# Autodesk Inventor assembly: Joining Plate T-Type for 4040 A
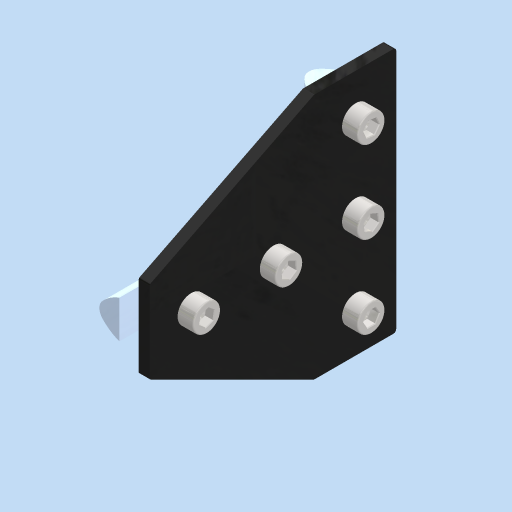
[picture p0: Inventor's stored thumbnail of the model, 512x512]
Saved by Autodesk Inventor 2023.2 (Build 272271000, 271)
## iProperties
Created: 2023-11-29
Part Number: Joining Plate T-Type for 4040 A
Document SubType Name: Assembly
Designer: Nils Bade
Author: Nils Bade
## Documents named in this file (5)
- C:\Users\nilsb\Documents\Inventor\Projektarbeit-Bade\RatRig_modified\Joining Plate T-Type for 4040 A - ItemNuts.iam
- C:\Users\nilsb\Documents\Inventor\Projektarbeit-Bade\RatRig_Standards\Joining Plate for 3030 - T - Black Anodized v2.ipt
- C:\Users\nilsb\Documents\Inventor\Projektarbeit-Bade\Schrauben\Cap Head Screw M6x12 v2.ipt
- C:\Users\nilsb\Documents\Inventor\Projektarbeit-Bade\ITEM\item_Nutenstein 8 - M6_0002623.ipt
- item_Nutenstein 8 - M6_0002623.ipt
## Components (11 placed, 3 different names)
1. Joining Plate for 3030 - T - Black Anodized v2:1 — Passend:1, Passend:2, Passend:3, Passend:4, Passend:5, Passend:6, Passend:7, Passend:8, Passend:9, Passend:10, Winkel:1, Winkel:2, Winkel:3, Winkel:4, Winkel:5, Passend:30, Passend:31, Passend:32, Passend:33, Passend:34
2. Cap Head Screw M6x12 v2:1 — Passend:1, Passend:7, Passend:26
3. Cap Head Screw M6x12 v2:2 — Passend:2, Passend:8, Passend:25
4. Cap Head Screw M6x12 v2:3 — Passend:3, Passend:6, Passend:29
5. Cap Head Screw M6x12 v2:4 — Passend:4, Passend:9, Passend:22, Passend:27
6. Cap Head Screw M6x12 v2:5 — Passend:5, Passend:10, Passend:21, Passend:28
7. item_Nutenstein 8 - M6_0002623:1 — Passend:28, Winkel:3, Passend:34
8. item_Nutenstein 8 - M6_0002623:2 — Passend:27, Winkel:2, Passend:31
9. item_Nutenstein 8 - M6_0002623:3 — Passend:29, Winkel:1, Passend:30
10. item_Nutenstein 8 - M6_0002623:4 — Passend:25, Winkel:4, Passend:32
11. item_Nutenstein 8 - M6_0002623:5 — Passend:26, Winkel:5, Passend:33
## Relationships (30: Mate 24, Angle 5, Flush 1)
- Passend:1 [Mate]: Joining Plate for 3030 - T - Black Anodized v2:1 ↔ Cap Head Screw M6x12 v2:1
- Passend:2 [Mate]: Joining Plate for 3030 - T - Black Anodized v2:1 ↔ Cap Head Screw M6x12 v2:2
- Passend:3 [Mate]: Joining Plate for 3030 - T - Black Anodized v2:1 ↔ Cap Head Screw M6x12 v2:3
- Passend:4 [Mate]: Joining Plate for 3030 - T - Black Anodized v2:1 ↔ Cap Head Screw M6x12 v2:4
- Passend:5 [Mate]: Joining Plate for 3030 - T - Black Anodized v2:1 ↔ Cap Head Screw M6x12 v2:5
- Passend:6 [Mate]: Joining Plate for 3030 - T - Black Anodized v2:1 ↔ Cap Head Screw M6x12 v2:3
- Passend:7 [Mate]: Joining Plate for 3030 - T - Black Anodized v2:1 ↔ Cap Head Screw M6x12 v2:1
- Passend:8 [Mate]: Joining Plate for 3030 - T - Black Anodized v2:1 ↔ Cap Head Screw M6x12 v2:2
- Passend:9 [Mate]: Joining Plate for 3030 - T - Black Anodized v2:1 ↔ Cap Head Screw M6x12 v2:4
- Passend:10 [Mate]: Joining Plate for 3030 - T - Black Anodized v2:1 ↔ Cap Head Screw M6x12 v2:5
- Passend:21 [Mate]: Cap Head Screw M6x12 v2:5
- Passend:22 [Mate]: Cap Head Screw M6x12 v2:4
- Passend:23 [Mate]
- Passend:24 [Mate]
- Fluchtend:1 [Flush] (-20 mm)
- Passend:25 [Mate]: Cap Head Screw M6x12 v2:2 ↔ item_Nutenstein 8 - M6_0002623:4
- Passend:26 [Mate]: Cap Head Screw M6x12 v2:1 ↔ item_Nutenstein 8 - M6_0002623:5
- Passend:27 [Mate]: Cap Head Screw M6x12 v2:4 ↔ item_Nutenstein 8 - M6_0002623:2
- Passend:28 [Mate]: Cap Head Screw M6x12 v2:5 ↔ item_Nutenstein 8 - M6_0002623:1
- Passend:29 [Mate]: Cap Head Screw M6x12 v2:3 ↔ item_Nutenstein 8 - M6_0002623:3
- Winkel:1 [Angle] (0 deg): Joining Plate for 3030 - T - Black Anodized v2:1 ↔ item_Nutenstein 8 - M6_0002623:3
- Winkel:2 [Angle] (0 deg): Joining Plate for 3030 - T - Black Anodized v2:1 ↔ item_Nutenstein 8 - M6_0002623:2
- Winkel:3 [Angle] (0 deg): Joining Plate for 3030 - T - Black Anodized v2:1 ↔ item_Nutenstein 8 - M6_0002623:1
- Winkel:4 [Angle] (0 deg): Joining Plate for 3030 - T - Black Anodized v2:1 ↔ item_Nutenstein 8 - M6_0002623:4
- Winkel:5 [Angle] (0 deg): Joining Plate for 3030 - T - Black Anodized v2:1 ↔ item_Nutenstein 8 - M6_0002623:5
- Passend:30 [Mate] (5.5 mm): Joining Plate for 3030 - T - Black Anodized v2:1 ↔ item_Nutenstein 8 - M6_0002623:3
- Passend:31 [Mate] (5.5 mm): Joining Plate for 3030 - T - Black Anodized v2:1 ↔ item_Nutenstein 8 - M6_0002623:2
- Passend:32 [Mate] (5.5 mm): Joining Plate for 3030 - T - Black Anodized v2:1 ↔ item_Nutenstein 8 - M6_0002623:4
- Passend:33 [Mate] (5.5 mm): Joining Plate for 3030 - T - Black Anodized v2:1 ↔ item_Nutenstein 8 - M6_0002623:5
- Passend:34 [Mate] (5.5 mm): Joining Plate for 3030 - T - Black Anodized v2:1 ↔ item_Nutenstein 8 - M6_0002623:1
